# Autodesk Inventor assembly: ASY GBK 2320 short wall shield 8
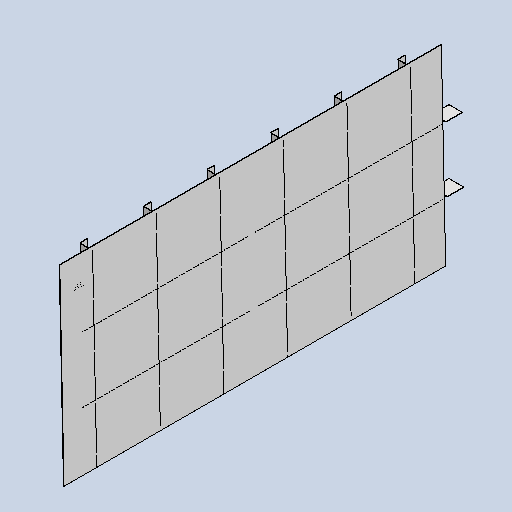
[picture p0: Inventor's stored thumbnail of the model, 512x512]
Saved by Autodesk Inventor 2026.2 (Build 302298010, 298A)
## iProperties
Created: 2026-05-07
Part Number: ASY GBK 2320 short wall shield 8
Document SubType Name: Assembly
Designer: pokla
Stock Number: 1321
Mass: 215512 g
Surface Area: 139105 cm^2
Volume: 27453.8 cm^3
Density: 7.85 g/cm^3
Author: admin
## Documents named in this file (6)
- C:\Users\admin\Documents\Inventor\GBK-Gubkinskiy\ASY GBK 2320 short wall shield 8.iam
- C:\Users\admin\Documents\Inventor\GBK-Gubkinskiy\GBK 0101 main rib.ipt
- C:\Users\admin\Documents\Inventor\GBK-Gubkinskiy\GBK 2321 shield 8.ipt
- C:\Users\admin\Documents\Inventor\GBK-Gubkinskiy\GBK 0302 stringer 7.ipt
- C:\Users\admin\Documents\Inventor\GBK-Gubkinskiy\GBK 0303 stringer 8.ipt
- C:\Users\admin\Documents\Inventor\GBK-Gubkinskiy\GBK 0301 third rib.ipt
## Components (11 placed, 4 different names)
1. GBK 0302 stringer 7.ipt:1 — Rigid:1, Rigid:4
2. GBK 0303 stringer 8.ipt:1 — Rigid:2, Rigid:3, Flush:3
3. GBK 2321 shield 8.ipt:1 — Mate:2, Mate:1, Flush:2, Flush:3
4. GBK 0303 stringer 8.ipt:2 — Rigid:3
5. GBK 0302 stringer 7.ipt:2 — Rigid:4
6. GBK 0301 third rib.ipt:1 — Mate:2, Mate:1, Rigid:2, Rigid:1
7. GBK 0301 third rib.ipt:2
8. GBK 0301 third rib.ipt:3
9. GBK 0301 third rib.ipt:4
10. GBK 0301 third rib.ipt:5
11. GBK 0301 third rib.ipt:6 — Mate:3, Mate:4
## Component patterns: (6 elements, first: GBK 0301 third rib.ipt:1)
## Relationships (10: Mate 4, WeldJoint 4, Flush 2)
- Mate:2: GBK 2321 shield 8.ipt:1 ↔ GBK 0301 third rib.ipt:1
- Mate:1: GBK 2321 shield 8.ipt:1 ↔ GBK 0301 third rib.ipt:1
- Rigid:2 [WeldJoint] (4 mm): GBK 0303 stringer 8.ipt:1 ↔ GBK 0301 third rib.ipt:1
- Rigid:1 [WeldJoint] (4 mm): GBK 0302 stringer 7.ipt:1 ↔ GBK 0301 third rib.ipt:1
- Rigid:3 [WeldJoint] (1 mm): GBK 0303 stringer 8.ipt:1 ↔ GBK 0303 stringer 8.ipt:2
- Rigid:4 [WeldJoint] (1 mm): GBK 0302 stringer 7.ipt:1 ↔ GBK 0302 stringer 7.ipt:2
- Mate:3: GBK 0301 third rib.ipt:6
- Mate:4: GBK 0301 third rib.ipt:6
- Flush:2: GBK 2321 shield 8.ipt:1
- Flush:3 (155 mm): GBK 0303 stringer 8.ipt:1 ↔ GBK 2321 shield 8.ipt:1
## Named parameters: основание_длина_нижнего = 200 mm, основание_длина_верхнего = 100 mm, стрингер_глубина_1 = 190.70056 mm, стрингер_глубина_2 = 179.35977 mm, стрингер_глубина_3 = 168.01899 mm, стрингер_глубина_4 = 156.6782 mm, стрингер_глубина_5 = 145.33742 mm, стрингер_глубина_6 = 133.99663 mm, стрингер_глубина_7 = 122.65585 mm, стрингер_глубина_8 = 111.31507 mm, Лист_ширина = 1480 mm, ребро_усилителей = 60 mm, паз_под_стрингер_глубина = 70 mm, паз_под_стрингер_толщина = 5 mm, отступ_от_пола_до_первого_стрингера = 410 mm, шаг_стрингеров = 500 mm, радиус_выреза_под_сварку = 30 mm, нахлест_шпангоутов_1_2 = 150 mm, нахлест_шпангоутов_2_3 = 120 mm, Стрингер_длина = 1489.5 mm, Лист_длина = 2980 mm, Шаг_шпангоутов = 496.66667 mm
